# Autodesk Inventor assembly: rev2 top short wall
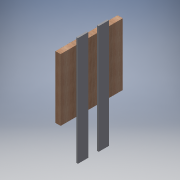
[picture p0: Inventor's stored thumbnail of the model, 180x180]
Saved by Autodesk Inventor 2017 (Build 210142000, 142)
## iProperties
Created: 2019-05-04
Part Number: rev2 top short wall
Document SubType Name: Assembly
Designer: Roman
Author: Roman
## Documents named in this file (3)
- C:\Users\Roman\Documents\CAD\enclosure rev1\rev2 short wall\rev2 top short wall.iam
- C:\Users\Roman\Documents\CAD\enclosure rev1\rev2 short wall\rev2 top short wall plane.ipt
- C:\Users\Roman\Documents\CAD\enclosure rev1\rev2 base\rev1 beam tube.ipt
## Components (3 placed, 2 different names)
1. rev2 top short wall plane:1 — Flush:1, Flush:2, Mate:1, Mate:2, Flush:3, Flush:4
2. rev1 beam tube:1 — Flush:2, Mate:2, Flush:4
3. rev1 beam tube:2 — Flush:1, Mate:1, Flush:3
## Relationships (6: Flush 4, Mate 2)
- Flush:1 (-101.6 mm): rev2 top short wall plane:1 ↔ rev1 beam tube:2
- Flush:2 (-101.6 mm): rev2 top short wall plane:1 ↔ rev1 beam tube:1
- Mate:1: rev2 top short wall plane:1 ↔ rev1 beam tube:2
- Mate:2: rev2 top short wall plane:1 ↔ rev1 beam tube:1
- Flush:3 (228.6 mm): rev2 top short wall plane:1 ↔ rev1 beam tube:2
- Flush:4 (228.6 mm): rev2 top short wall plane:1 ↔ rev1 beam tube:1
